# Autodesk Inventor assembly: Test
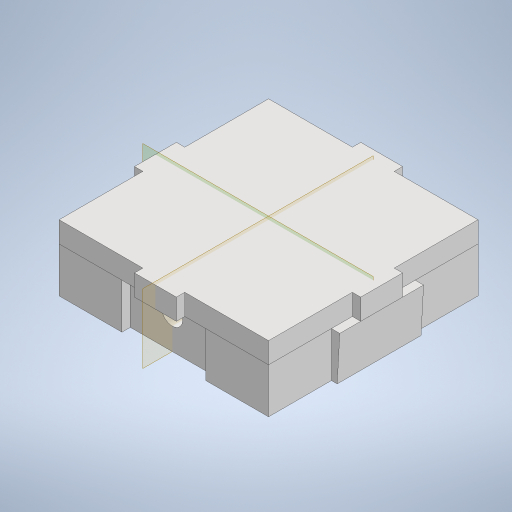
[picture p0: Inventor's stored thumbnail of the model, 512x512]
Saved by Autodesk Inventor 2024 (Build 280153000, 153)
## iProperties
Created: 2023-11-08
Part Number: Test
Document SubType Name: Assembly
Designer: Piter
Author: Piter
## Documents named in this file (5)
- C:\Users\Piter\OneDrive\Pulpit\Modele\My projects\My-3D-printing-projects\Prezent\Test.iam
- C:\Users\Piter\OneDrive\Pulpit\Modele\My projects\My-3D-printing-projects\Prezent\test_up.ipt
- C:\Users\Piter\OneDrive\Pulpit\Modele\My projects\My-3D-printing-projects\Prezent\Pokrywka.ipt
- C:\Users\Piter\OneDrive\Pulpit\Modele\My projects\My-3D-printing-projects\Prezent\Pin.ipt
- C:\Users\Piter\OneDrive\Pulpit\Modele\My projects\My-3D-printing-projects\Prezent\opaska_test.ipt
## Components (4 placed, 4 different names)
1. test_up:1 — Mate:1, Mate:2, Mate:3, Mate:4, Mate:7
2. Pokrywka:1 — Mate:1, Mate:2, Mate:4, Mate:6
3. Pin:1 — Mate:3, Mate:5
4. opaska_test:1 — Mate:5, Mate:6, Mate:7
## Relationships (7: Mate 7)
- Mate:1: test_up:1 ↔ Pokrywka:1
- Mate:2: test_up:1 ↔ Pokrywka:1
- Mate:3: test_up:1 ↔ Pin:1
- Mate:4: test_up:1 ↔ Pokrywka:1
- Mate:5: Pin:1 ↔ opaska_test:1
- Mate:6: Pokrywka:1 ↔ opaska_test:1
- Mate:7: test_up:1 ↔ opaska_test:1
